# Autodesk Inventor assembly: Stage2
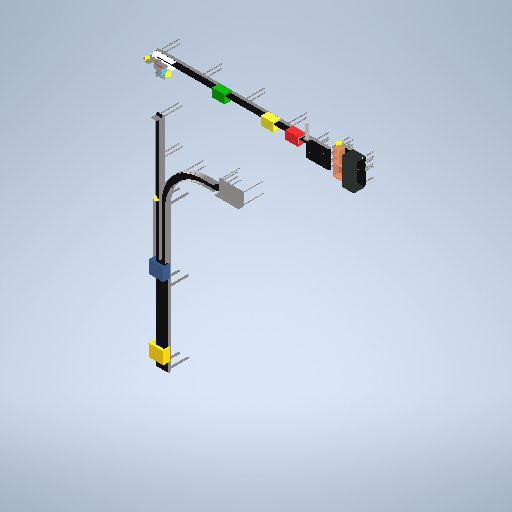
[picture p0: Inventor's stored thumbnail of the model, 512x512]
Saved by Autodesk Inventor 2025.1 (Build 291241000, 241)
## iProperties
Created: 2025-02-26
Part Number: Stage2
Document SubType Name: Assembly
Designer: yovan
Author: yovan
## Documents named in this file (18)
- C:\Users\yovan\Desktop\APM\ausol-apm.github.io\project\Design and simulation\Inventor\NXModeling\Stage2.iam
- C:\Users\yovan\Desktop\APM\ausol-apm.github.io\project\Design and simulation\Inventor\NXModeling\Assembler.ipt
- C:\Users\yovan\Desktop\APM\ausol-apm.github.io\project\Design and simulation\Inventor\NXModeling\ConveyorsStage2-3.ipt
- C:\Users\yovan\Desktop\APM\ausol-apm.github.io\project\Design and simulation\Inventor\Modelado juguetes\Barco\EnsamblajeBarco.iam
- C:\Users\yovan\Desktop\APM\ausol-apm.github.io\project\Design and simulation\Inventor\Modelado juguetes\Barco\Piezabarcosuperior.ipt
- C:\Users\yovan\Desktop\APM\ausol-apm.github.io\project\Design and simulation\Inventor\Modelado juguetes\Barco\PiezaEjeTimon.ipt
- C:\Users\yovan\Desktop\APM\ausol-apm.github.io\project\Design and simulation\Inventor\Modelado juguetes\Barco\PiezaTimon.ipt
- C:\Users\yovan\Desktop\APM\ausol-apm.github.io\project\Design and simulation\Inventor\Modelado juguetes\Moto\EnsamblajeMoto.iam
- C:\Users\yovan\Desktop\APM\ausol-apm.github.io\project\Design and simulation\Inventor\Modelado juguetes\Moto\Llanta.ipt
- C:\Users\yovan\Desktop\APM\ausol-apm.github.io\project\Design and simulation\Inventor\NXModeling\Sensor.ipt
- C:\Users\yovan\Desktop\APM\ausol-apm.github.io\project\Design and simulation\Inventor\Modelado juguetes\Casa\TechoCasa.ipt
- C:\Users\yovan\Desktop\APM\ausol-apm.github.io\project\Design and simulation\Inventor\Modelado juguetes\Casa\EnsamblajeCasa.iam
- C:\Users\yovan\Desktop\APM\ausol-apm.github.io\project\Design and simulation\Inventor\NXModeling\PneumaticActuator\PneummaticActuator.iam
- C:\Users\yovan\Desktop\APM\ausol-apm.github.io\project\Design and simulation\Inventor\NXModeling\Caja grande.ipt
- C:\Users\yovan\Desktop\APM\ausol-apm.github.io\project\Design and simulation\Inventor\NXModeling\Caja pequeña.ipt
- C:\Users\yovan\Desktop\APM\ausol-apm.github.io\project\Design and simulation\Inventor\NXModeling\ConveyorS&F.ipt
- C:\Users\yovan\Desktop\APM\ausol-apm.github.io\project\Design and simulation\Inventor\NXModeling\BiggerPneumatic\biggerAct.iam
- C:\Users\yovan\Desktop\APM\ausol-apm.github.io\project\Design and simulation\Inventor\NXModeling\Camera.ipt
## Components (37 placed, 17 different names)
1. Assembler:1 — Flush:1, Mate:1, Tangent:1, Flush:2, Mate:2, Mate:3, Mate:4, Tangent:2, Mate:5, Tangent:3, Mate:6, Mate:7, Mate:8, Mate:9, Insert:2, Mate:10, Insert:3, Insert:4, Insert:5, Insert:6, Mate:11, Mate:12, Insert:7, Mate:13, Mate:14, Mate:15, Insert:8, Mate:16, Mate:17, Mate:18, Mate:19, Mate:20, Mate:21, Mate:22, Mate:23, Mate:24, Mate:25, Mate:26, Mate:27, Mate:28, Mate:29, Mate:30, Mate:39, Mate:40
2. ConveyorsStage2-3:1 — Flush:1, Mate:1, Tangent:1, Mate:31, Tangent:4, Flush:3, Tangent:5, Mate:32, Flush:4, Tangent:6, Mate:33, Flush:35, Tangent:7, Tangent:8, Flush:36, Mate:34, Mate:35, Mate:36, Mate:37, Mate:38, Mate:41
3. EnsamblajeBarco:1 [sub-assembly] — Flush:2, Mate:2
4. Piezabarcosuperior:1 — Mate:3, Mate:4
5. PiezaEjeTimon:1 — Insert:1
6. PiezaTimon:1 — Insert:1, Tangent:2, Mate:5, Tangent:3
7. EnsamblajeMoto:1 [sub-assembly] — Mate:6, Mate:7
8. Llanta:1 — Mate:8
9. Llanta:2 — Mate:9
10. Sensor:1 — Insert:2
11. Sensor:2 — Mate:10
12. Sensor:3 — Insert:3
13. Sensor:4 — Insert:4
14. Sensor:5 — Insert:5
15. Sensor:6 — Insert:6
16. TechoCasa:1 — Mate:11, Mate:12
17. Sensor:7 — Insert:7
18. EnsamblajeCasa:1 [sub-assembly] — Mate:13, Mate:14, Mate:15
19. Sensor:8 — Insert:8
20. PneummaticActuator:1 [sub-assembly] — Mate:16, Mate:17
21. PneummaticActuator:2 [sub-assembly] — Mate:18, Mate:21
22. PneummaticActuator:3 [sub-assembly] — Mate:19, Mate:20
23. PneummaticActuator:4 [sub-assembly] — Mate:24, Mate:25
24. PneummaticActuator:5 [sub-assembly] — Mate:30
25. PneummaticActuator:6 [sub-assembly] — Mate:22, Mate:23
26. PneummaticActuator:7 [sub-assembly] — Mate:26
27. PneummaticActuator:9 [sub-assembly] — Mate:27, Mate:28
28. PneummaticActuator:10 [sub-assembly] — Mate:29
29. Caja grande:1 — Mate:31, Tangent:4, Flush:3
30. Caja pequeña:1 — Tangent:5, Mate:32, Flush:4
31. Caja pequeña:2 — Tangent:6, Mate:33, Flush:35
32. ConveyorS&F:1 — Tangent:7, Tangent:8, Flush:36
33. biggerAct:1 [sub-assembly] — Mate:34, Mate:35
34. Camera:1 — Mate:36, Mate:37, Mate:38
35. Sensor:9 — Mate:39
36. Sensor:10 — Mate:40
37. Sensor:11 — Mate:41
## Relationships (63: Mate 41, Tangent 8, Insert 8, Flush 6)
- Flush:1 (-135 mm): Assembler:1 ↔ ConveyorsStage2-3:1
- Mate:1 (300 mm): Assembler:1 ↔ ConveyorsStage2-3:1
- Tangent:1 (-120 mm): Assembler:1 ↔ ConveyorsStage2-3:1
- Flush:2 (-25 mm): Assembler:1 ↔ EnsamblajeBarco:1
- Mate:2: Assembler:1 ↔ EnsamblajeBarco:1
- Mate:3: Assembler:1 ↔ Piezabarcosuperior:1
- Mate:4: Assembler:1 ↔ Piezabarcosuperior:1
- Insert:1: PiezaEjeTimon:1 ↔ PiezaTimon:1
- Tangent:2: Assembler:1 ↔ PiezaTimon:1
- Mate:5 (2 mm): Assembler:1 ↔ PiezaTimon:1
- Tangent:3 (2.5 mm): Assembler:1 ↔ PiezaTimon:1
- Mate:6: Assembler:1 ↔ EnsamblajeMoto:1
- Mate:7: Assembler:1 ↔ EnsamblajeMoto:1
- Mate:8 (1.5 mm): Assembler:1 ↔ Llanta:1
- Mate:9 (1.5 mm): Assembler:1 ↔ Llanta:2
- Insert:2 (-10 mm): Assembler:1 ↔ Sensor:1
- Mate:10: Assembler:1 ↔ Sensor:2
- Insert:3 (-5 mm): Assembler:1 ↔ Sensor:3
- Insert:4 (-7 mm): Assembler:1 ↔ Sensor:4
- Insert:5 (-4 mm): Assembler:1 ↔ Sensor:5
- Insert:6 (-5 mm): Assembler:1 ↔ Sensor:6
- Mate:11: Assembler:1 ↔ TechoCasa:1
- Mate:12: Assembler:1 ↔ TechoCasa:1
- Insert:7 (-10 mm): Assembler:1 ↔ Sensor:7
- Mate:13: Assembler:1 ↔ EnsamblajeCasa:1
- Mate:14 (10 mm): Assembler:1 ↔ EnsamblajeCasa:1
- Mate:15: Assembler:1 ↔ EnsamblajeCasa:1
- Insert:8 (-7 mm): Assembler:1 ↔ Sensor:8
- Mate:16: Assembler:1 ↔ PneummaticActuator:1
- Mate:17 (10 mm): Assembler:1 ↔ PneummaticActuator:1
- Mate:18: Assembler:1 ↔ PneummaticActuator:2
- Mate:19: Assembler:1 ↔ PneummaticActuator:3
- Mate:20 (10 mm): Assembler:1 ↔ PneummaticActuator:3
- Mate:21 (10 mm): Assembler:1 ↔ PneummaticActuator:2
- Mate:22: Assembler:1 ↔ PneummaticActuator:6
- Mate:23 (15 mm): Assembler:1 ↔ PneummaticActuator:6
- Mate:24: Assembler:1 ↔ PneummaticActuator:4
- Mate:25 (10 mm): Assembler:1 ↔ PneummaticActuator:4
- Mate:26: Assembler:1 ↔ PneummaticActuator:7
- Mate:27: Assembler:1 ↔ PneummaticActuator:9
- Mate:28 (9 mm): Assembler:1 ↔ PneummaticActuator:9
- Mate:29: Assembler:1 ↔ PneummaticActuator:10
- Mate:30: Assembler:1 ↔ PneummaticActuator:5
- Mate:31: ConveyorsStage2-3:1 ↔ Caja grande:1
- Tangent:4 (-120 mm): ConveyorsStage2-3:1 ↔ Caja grande:1
- Flush:3: ConveyorsStage2-3:1 ↔ Caja grande:1
- Tangent:5 (-120 mm): ConveyorsStage2-3:1 ↔ Caja pequeña:1
- Mate:32: ConveyorsStage2-3:1 ↔ Caja pequeña:1
- Flush:4: ConveyorsStage2-3:1 ↔ Caja pequeña:1
- Tangent:6 (-120 mm): ConveyorsStage2-3:1 ↔ Caja pequeña:2
- Mate:33: ConveyorsStage2-3:1 ↔ Caja pequeña:2
- Flush:35: ConveyorsStage2-3:1 ↔ Caja pequeña:2
- Tangent:7 (2000 mm): ConveyorsStage2-3:1 ↔ ConveyorS&F:1
- Tangent:8 (-250 mm): ConveyorsStage2-3:1 ↔ ConveyorS&F:1
- Flush:36: ConveyorsStage2-3:1 ↔ ConveyorS&F:1
- Mate:34: ConveyorsStage2-3:1 ↔ biggerAct:1
- Mate:35: ConveyorsStage2-3:1 ↔ biggerAct:1
- Mate:36 (-30 mm): ConveyorsStage2-3:1 ↔ Camera:1
- Mate:37: ConveyorsStage2-3:1 ↔ Camera:1
- Mate:38: ConveyorsStage2-3:1 ↔ Camera:1
- Mate:39: Assembler:1 ↔ Sensor:9
- Mate:40: Assembler:1 ↔ Sensor:10
- Mate:41: ConveyorsStage2-3:1 ↔ Sensor:11
